# Autodesk Inventor assembly: КВ33.044.400 - Сборка деражтеля катка 6 мм
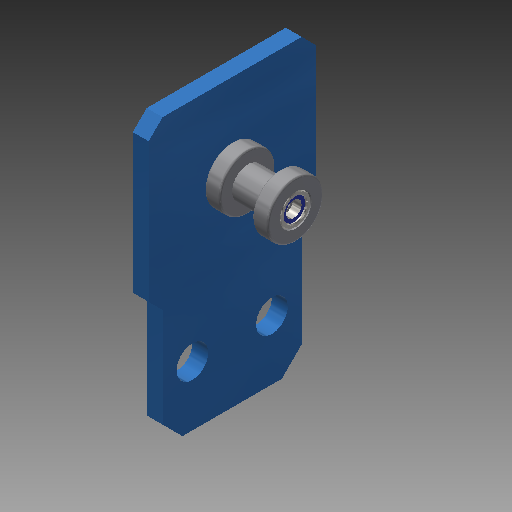
[picture p0: Inventor's stored thumbnail of the model, 512x512]
Saved by Autodesk Inventor 2019 (Build 230136000, 136)
## iProperties
Created: 2019-07-17
Part Number: КВ33.044.400 - Сборка деражтеля катка 6 мм
Material: Типовые
Document SubType Name: Assembly
Designer: Петров Иван
Author: Петров Иван
## Documents named in this file (3)
- C:\Users\user\Documents\Kvantoriada2019\optimal_gripper\hardware\КВ33.044.700 - Сборка деражтеля катка 6 мм.iam
- C:\Users\user\Documents\Kvantoriada2019\optimal_gripper\hardware\КВ33.044.701 - Держатель катка 6 мм.ipt
- C:\Users\user\Documents\Kvantoriada2019\optimal_gripper\hardware\КВ33.044.800 - Шкив плоский Makeblock сборка.iam
## Components (2 placed, 2 different names)
1. КВ33.044.701 - Держатель катка 6 мм:1 — Совмещение:1, Совмещение:2
2. КВ33.044.800 - Шкив плоский Makeblock сборка:1 [sub-assembly] — Совмещение:1, Совмещение:2
## Relationships (2: Mate 2)
- Совмещение:1 [Mate]: КВ33.044.701 - Держатель катка 6 мм:1 ↔ КВ33.044.800 - Шкив плоский Makeblock сборка:1
- Совмещение:2 [Mate]: КВ33.044.701 - Держатель катка 6 мм:1 ↔ КВ33.044.800 - Шкив плоский Makeblock сборка:1
